# Autodesk Inventor assembly: ASY Workshop big
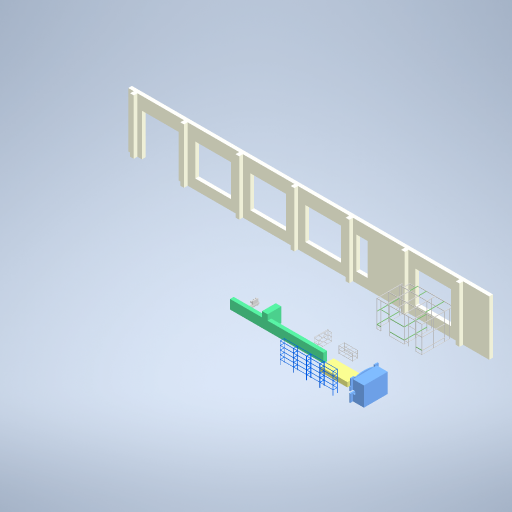
[picture p0: Inventor's stored thumbnail of the model, 512x512]
Saved by Autodesk Inventor 2024.2 (Build 282272000, 272)
## iProperties
Created: 2024-04-06
Part Number: ASY Workshop big
Document SubType Name: Assembly
Designer: admin
Author: admin
## Documents named in this file (10)
- C:\Users\admin\My Drive (bigstupidbeast@gmail.com)\Inventor\Workshop\ASY Workshop big.iam
- C:\Users\admin\My Drive (bigstupidbeast@gmail.com)\Inventor\Workshop\Structures\Wall 5.ipt
- C:\Users\admin\My Drive (bigstupidbeast@gmail.com)\Inventor\Workshop\оборудование\compressor.ipt
- C:\Users\admin\My Drive (bigstupidbeast@gmail.com)\Inventor\Workshop\оборудование\гибочный пресс\Hydraulic Sheet Metal Bending Machine PBH-135T3200 3000.ipt
- C:\Users\admin\My Drive (bigstupidbeast@gmail.com)\Inventor\Workshop\Part2.ipt
- C:\Users\admin\My Drive (bigstupidbeast@gmail.com)\Inventor\Workshop\rack\Rack 2\ASY rack 2.iam
- C:\Users\admin\My Drive (bigstupidbeast@gmail.com)\Inventor\Workshop\roller conveyor\roller conveyor 1\ASY roller conveyor 1.iam
- C:\Users\admin\My Drive (bigstupidbeast@gmail.com)\Inventor\Workshop\Table wheel\ASY table wheel 1.iam
- C:\Users\admin\My Drive (bigstupidbeast@gmail.com)\Inventor\Workshop\pallet dummy.ipt
- C:\Users\admin\My Drive (bigstupidbeast@gmail.com)\Inventor\Workshop\ASY WRS АБК.iam
## Components (12 placed, 9 different names)
1. Wall 5:1 — Flush:1, Flush:5, Flush:6
2. compressor:1
3. Hydraulic Sheet Metal Bending Machine PBH-135T3200 3000:1 — Flush:1
4. Part2:1 — Flush:2
5. ASY roller conveyor 1:1 [sub-assembly] — Mate:7
6. ASY table wheel 1:1 [sub-assembly] — Mate:6
7. pallet dummy:1 — Flush:3
8. ASY WRS АБК:1 [sub-assembly] — Flush:4, Flush:5, Flush:6
9. ASY rack 2:1 [sub-assembly] — Mate:4
10. ASY rack 2:2 [sub-assembly]
11. ASY rack 2:3 [sub-assembly]
12. ASY rack 2:4 [sub-assembly]
## Component patterns: (4 elements, first: ASY rack 2:1)
## Relationships (9: Flush 6, Mate 3)
- Flush:1: Wall 5:1 ↔ Hydraulic Sheet Metal Bending Machine PBH-135T3200 3000:1
- Flush:2: Part2:1
- Mate:4: ASY rack 2:1
- Flush:3: pallet dummy:1
- Flush:4: ASY WRS АБК:1
- Mate:6: ASY table wheel 1:1
- Mate:7: ASY roller conveyor 1:1
- Flush:5: Wall 5:1 ↔ ASY WRS АБК:1
- Flush:6 (120 mm): Wall 5:1 ↔ ASY WRS АБК:1
